# Autodesk Inventor assembly: [总]惯性筛总装配
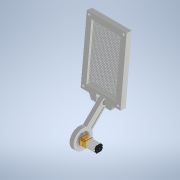
[picture p0: Inventor's stored thumbnail of the model, 180x180]
Saved by Autodesk Inventor 2022 (Build 260153000, 153)
## iProperties
Created: 2022-05-21
Part Number: [总]惯性筛总装配
Document SubType Name: Assembly
Designer: zhcne
Author: zhcne
## Documents named in this file (3)
- E:\Engineering_Development\SchoolProjects\2022_5_18_惯性筛_机电一体化课程设计\inertiascreen_curriculumdesign\3.Model\2.3D_Simulation\[总]惯性筛总装配.iam
- E:\Engineering_Development\SchoolProjects\2022_5_18_惯性筛_机电一体化课程设计\inertiascreen_curriculumdesign\3.Model\2.3D_Simulation\惯性筛筛网装配.iam
- E:\Engineering_Development\SchoolProjects\2022_5_18_惯性筛_机电一体化课程设计\inertiascreen_curriculumdesign\3.Model\2.3D_Simulation\惯性筛偏心轮装配.iam
## Components (2 placed, 2 different names)
1. 惯性筛筛网装配:1 [sub-assembly] — 配合:1, 配合:2
2. 惯性筛偏心轮装配:1 [sub-assembly] — 配合:1, 配合:2, 配合:3
## Relationships (3: Mate 3)
- 配合:1 [Mate] (4 mm): 惯性筛筛网装配:1 ↔ 惯性筛偏心轮装配:1
- 配合:2 [Mate]: 惯性筛筛网装配:1 ↔ 惯性筛偏心轮装配:1
- 配合:3 [Mate]: 惯性筛偏心轮装配:1
